# Autodesk Inventor assembly: camera_and_lens
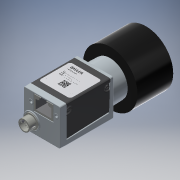
[picture p0: Inventor's stored thumbnail of the model, 180x180]
Saved by Autodesk Inventor 2018 (Build 220112000, 112)
## iProperties
Created: 2019-07-26
Part Number: camera_and_lens
Document SubType Name: Assembly
Designer: Jasper
Author: Jasper
## Documents named in this file (3)
- C:\Users\jaspe\bitbots_hardware\camera\camera_and_lens.iam
- C:\Users\jaspe\bitbots_hardware\camera\lens.ipt
- C:\Users\jaspe\bitbots_hardware\camera\Basler ace GigE C-Mount v01.ipt
## Components (2 placed, 2 different names)
1. lens:1 — Mate:2, Mate:3
2. Basler ace GigE C-Mount v01:1 — Mate:1, Mate:2, Mate:3
## Relationships (3: Mate 3)
- Mate:1: Basler ace GigE C-Mount v01:1
- Mate:2: lens:1 ↔ Basler ace GigE C-Mount v01:1
- Mate:3: lens:1 ↔ Basler ace GigE C-Mount v01:1
